# Autodesk Inventor assembly: Neuronexus
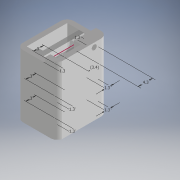
[picture p0: Inventor's stored thumbnail of the model, 180x180]
Saved by Autodesk Inventor 2020 (Build 240168000, 168)
## iProperties
Created: 2020-02-24
Part Number: Neuronexus
Document SubType Name: Assembly
Designer: Knowblesse
Author: Knowblesse
## Documents named in this file (9)
- C:\VCF\Microdrive\Neuronexus\Neuronexus.iam
- C:\VCF\Microdrive\Neuronexus\Bot.ipt
- C:\VCF\Microdrive\Neuronexus\Mid.ipt
- C:\VCF\Microdrive\Neuronexus\Screw.ipt
- C:\VCF\Microdrive\Neuronexus\Top.ipt
- C:\VCF\Microdrive\Neuronexus\19G_Pillar.ipt
- C:\VCF\Microdrive\Neuronexus\Case.ipt
- C:\VCF\Microdrive\Neuronexus\Case_Top.ipt
- C:\VCF\Microdrive\Neuronexus\Case_Cover.ipt
## Components (9 placed, 8 different names)
1. Bot:1 — 강체:1, 강체:2, 강체:3
2. Mid:1 — 원통형:1, 원통형:2
3. Screw:1 — 회전:1
4. Top:1 — 원통형:3, 원통형:4, 회전:1, 메이트:1
5. 19G_Pillar:1 — 강체:2, 원통형:1, 원통형:4, 메이트:1
6. 19G_Pillar:2 — 강체:1, 원통형:2, 원통형:3
7. Case:1 — 강체:3, 강체:4
8. Case_Top:1
9. Case_Cover:1 — 강체:4
## Relationships (10: WeldJoint 4, CylindricalJoint 4, RevoluteJoint 1, Mate 1)
- 강체:1 [WeldJoint]: Bot:1 ↔ 19G_Pillar:2
- 강체:2 [WeldJoint]: Bot:1 ↔ 19G_Pillar:1
- 원통형:1 [CylindricalJoint]: Mid:1 ↔ 19G_Pillar:1
- 원통형:2 [CylindricalJoint]: Mid:1 ↔ 19G_Pillar:2
- 원통형:3 [CylindricalJoint]: Top:1 ↔ 19G_Pillar:2
- 원통형:4 [CylindricalJoint]: Top:1 ↔ 19G_Pillar:1
- 회전:1 [RevoluteJoint]: Screw:1 ↔ Top:1
- 강체:3 [WeldJoint]: Bot:1 ↔ Case:1
- 메이트:1 [Mate]: Top:1 ↔ 19G_Pillar:1
- 강체:4 [WeldJoint]: Case:1 ↔ Case_Cover:1
